# Autodesk Inventor assembly: pistonassembly
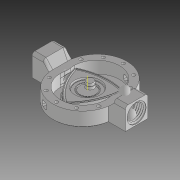
[picture p0: Inventor's stored thumbnail of the model, 180x180]
Saved by Autodesk Inventor 2020 (Build 240168000, 168)
## iProperties
Created: 2020-11-25
Part Number: pistonassembly
Document SubType Name: Assembly
Designer: DDeGo
Author: DDeGo
## Documents named in this file (9)
- C:\Users\DDeGo\Documents\Drew\Projects\AirWankelEngine\cad\EngineAssembly.iam
- C:\Users\DDeGo\Documents\Drew\Projects\AirWankelEngine\cad\housing.ipt
- C:\Users\DDeGo\Documents\Drew\Projects\AirWankelEngine\cad\piston.ipt
- C:\Users\DDeGo\Documents\Drew\Projects\AirWankelEngine\cad\camshaft.ipt
- C:\Users\DDeGo\Documents\Drew\Projects\AirWankelEngine\cad\6701 bearing.ipt
- C:\Users\DDeGo\Documents\Drew\Projects\AirWankelEngine\cad\MR85 bearing.ipt
- C:\Users\DDeGo\Documents\Drew\Projects\AirWankelEngine\cad\oring_5p5x7p5.ipt
- C:\Users\DDeGo\Documents\Drew\Projects\AirWankelEngine\cad\6mm bb.ipt
- C:\Users\DDeGo\Documents\Drew\Projects\AirWankelEngine\cad\housingPlate.ipt
## Components (10 placed, 8 different names)
1. housing:1 — Mate:1, Mate:4, Mate:14, Mate:21, Mate:22, Mate:23
2. piston:1 — Mate:1, Mate:2, Mate:12
3. camshaft:1 — Mate:4, Mate:5, Mate:8, Mate:13
4. 6701 bearing:1 — Mate:2, Mate:5, Mate:12
5. MR85 bearing:1 — Mate:8, Mate:13, Mate:14
6. oring_5p5x7p5:1
7. oring_5p5x7p5:2
8. 6mm bb:1
9. housingPlate:1 — Mate:21, Mate:22, Mate:23
10. 6mm bb:2
## Relationships (11: Mate 11)
- Mate:1: housing:1 ↔ piston:1
- Mate:2: piston:1 ↔ 6701 bearing:1
- Mate:4: housing:1 ↔ camshaft:1
- Mate:5: camshaft:1 ↔ 6701 bearing:1
- Mate:8: camshaft:1 ↔ MR85 bearing:1
- Mate:12: piston:1 ↔ 6701 bearing:1
- Mate:13: camshaft:1 ↔ MR85 bearing:1
- Mate:14: housing:1 ↔ MR85 bearing:1
- Mate:21: housing:1 ↔ housingPlate:1
- Mate:22: housing:1 ↔ housingPlate:1
- Mate:23: housing:1 ↔ housingPlate:1
